# Autodesk Inventor assembly: XcrLeft
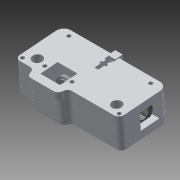
[picture p0: Inventor's stored thumbnail of the model, 180x180]
Saved by Autodesk Inventor 2013 (Build 170138000, 138)
## iProperties
Created: 2015-01-14
Part Number: XcrLeft
Document SubType Name: Assembly
Designer: dzban
Author: dzban
## Documents named in this file (9)
- D:\PIRX\Artisan\OPENSOURCE\XCars\XcrLeft.iam
- D:\PIRX\Artisan\OPENSOURCE\XCars\XcrLeft_b.ipt
- D:\PIRX\Artisan\OPENSOURCE\XCars\XcrLeft_a.ipt
- D:\PIRX\Artisan\OPENSOURCE\StockComponents\LM08UU.ipt
- D:\PIRX\Artisan\OPENSOURCE\XCars\XcrLeft_c.ipt
- D:\PIRX\Artisan\OPENSOURCE\XCars\XcrLeftPulleyShaft.ipt
- D:\PIRX\Artisan\OPENSOURCE\XCars\XcrLeftBeltTensioner.ipt
- D:\PIRX\Artisan\OPENSOURCE\XCars\XcrLeftPulleyAlu.ipt
- D:\PIRX\Artisan\OPENSOURCE\StockComponents\625ZZ_bearing.ipt
## Components (11 placed, 8 different names)
1. XcrLeft_a:1 — Mate:1, Tangent:1, Tangent:2, Mate:2, Tangent:3, Tangent:4, Insert:1, Insert:2, Mate:3, Tangent:5, Flush:1, Mate:4
2. LM08UU:1 — Mate:2, Tangent:3, Tangent:4
3. LM08UU:2 — Mate:1, Tangent:1, Tangent:2
4. XcrLeft_c:1 — Insert:3, Insert:4, Insert:5, Insert:6
5. XcrLeft_c:2 — Insert:1, Insert:2, Insert:3, Insert:4
6. XcrLeft_b:1 — Insert:5, Insert:6, Tangent:6
7. XcrLeftPulleyShaft:1 — Insert:7
8. XcrLeftBeltTensioner:1 — Flush:1, Mate:4
9. XcrLeftPulleyAlu:1 — Insert:7, Insert:8, Insert:9
10. 625ZZ_bearing:1 — Insert:9
11. 625ZZ_bearing:2 — Insert:8, Mate:3, Tangent:5, Tangent:6
## Relationships (20: Insert 9, Tangent 6, Mate 4, Flush 1)
- Mate:1: XcrLeft_a:1 ↔ LM08UU:2
- Tangent:1: XcrLeft_a:1 ↔ LM08UU:2
- Tangent:2: XcrLeft_a:1 ↔ LM08UU:2
- Mate:2: XcrLeft_a:1 ↔ LM08UU:1
- Tangent:3: XcrLeft_a:1 ↔ LM08UU:1
- Tangent:4: XcrLeft_a:1 ↔ LM08UU:1
- Insert:1: XcrLeft_a:1 ↔ XcrLeft_c:2
- Insert:2: XcrLeft_a:1 ↔ XcrLeft_c:2
- Insert:3: XcrLeft_c:1 ↔ XcrLeft_c:2
- Insert:4: XcrLeft_c:1 ↔ XcrLeft_c:2
- Insert:5: XcrLeft_c:1 ↔ XcrLeft_b:1
- Insert:6: XcrLeft_c:1 ↔ XcrLeft_b:1
- Insert:7 (-14.7 mm): XcrLeftPulleyShaft:1 ↔ XcrLeftPulleyAlu:1
- Insert:8: XcrLeftPulleyAlu:1 ↔ 625ZZ_bearing:2
- Insert:9: XcrLeftPulleyAlu:1 ↔ 625ZZ_bearing:1
- Mate:3: XcrLeft_a:1 ↔ 625ZZ_bearing:2
- Tangent:5: XcrLeft_a:1 ↔ 625ZZ_bearing:2
- Tangent:6: XcrLeft_b:1 ↔ 625ZZ_bearing:2
- Flush:1: XcrLeft_a:1 ↔ XcrLeftBeltTensioner:1
- Mate:4: XcrLeft_a:1 ↔ XcrLeftBeltTensioner:1
